# Autodesk Inventor assembly: 조립품1
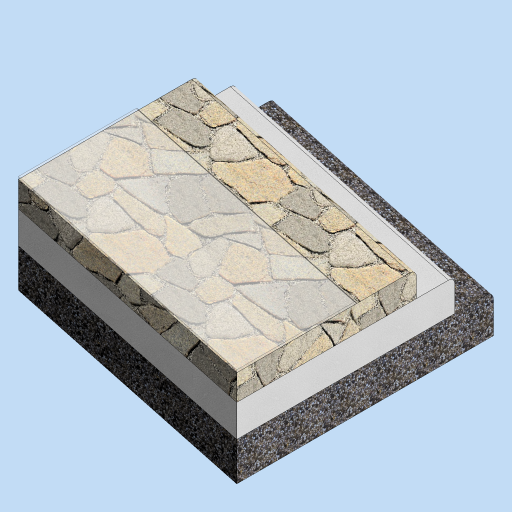
[picture p0: Inventor's stored thumbnail of the model, 512x512]
Saved by Autodesk Inventor 2024.1 (Build 281209000, 209)
## iProperties
Created: 2024-01-18
Part Number: 조립품1
Document SubType Name: Assembly
Designer: likek
Author: likek
## Documents named in this file (4)
- C:\Users\likek\OneDrive\바탕 화면\조립품1.iam
- C:\Users\likek\OneDrive\바탕 화면\부품1.ipt
- C:\Users\likek\OneDrive\바탕 화면\부품2.ipt
- C:\Users\likek\OneDrive\바탕 화면\부품3.ipt
## Components (3 placed, 3 different names)
1. 부품1:1 — 강체:1, 강체:2
2. 부품2:1 — 강체:1
3. 부품3:1 — 강체:2
## Relationships (2: WeldJoint 2)
- 강체:1 [WeldJoint]: 부품1:1 ↔ 부품2:1
- 강체:2 [WeldJoint]: 부품1:1 ↔ 부품3:1
